# Autodesk Inventor assembly: frameortho
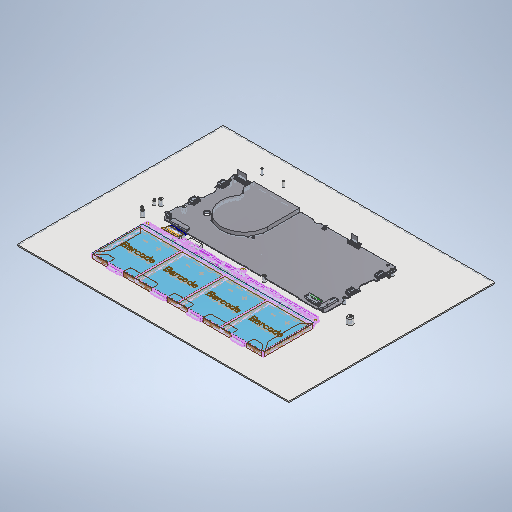
[picture p0: Inventor's stored thumbnail of the model, 512x512]
Saved by Autodesk Inventor 2025 (Build 290162010, 162A)
## iProperties
Created: 2026-01-15
Part Number: frameortho
Document SubType Name: Assembly
Designer: 200481997
Author: 200481997
## Documents named in this file (4)
- C:\Users\200481997\Documents\GitHub\frameortho\CAD\frameergo.iam
- C:\Users\200481997\Documents\GitHub\frameortho\CAD\Imports\Battery\FWKNAQ9_G01_20210911\Framework BatteryFWKNAQ9_G01_20210911.ipt
- C:\Users\200481997\Documents\GitHub\frameortho\CAD\chassis.ipt
- C:\Users\200481997\Documents\GitHub\frameortho\CAD\Imports\Motherboard\Framework Mobo\Framework Mobo.ipt
## Components (3 placed, 3 different names)
1. Framework Battery
2. chassis:1 — Mate:1, Mate:2
3. Framework Mobo:1 — Mate:1, Mate:2
## Relationships (2: Mate 2)
- Mate:1: chassis:1 ↔ Framework Mobo:1
- Mate:2: chassis:1 ↔ Framework Mobo:1
